# Autodesk Inventor assembly: Assembly_Matchboxscope_injectionmolded_holo
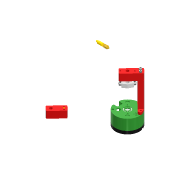
[picture p0: Inventor's stored thumbnail of the model, 180x180]
Saved by Autodesk Inventor 2022 (Build 260153000, 153)
## iProperties
Created: 2023-04-12
Part Number: Assembly_Matchboxscope_injectionmolded_holo
Document SubType Name: Assembly
Designer: diederichbenedict
Author: diederichbenedict
## Documents named in this file (11)
- C:\Users\diederichbenedict\Dropbox\Dokumente\Promotion\PROJECTS\Matchboxscope\INVENTOR\RELEASE\InjectionMolded\Assembly_Matchboxscope_injectionmolded_holo.iam
- C:\Users\diederichbenedict\Dropbox\Dokumente\Promotion\PROJECTS\Matchboxscope\INVENTOR\RELEASE\InjectionMolded\IM_Matchboxscope_base.ipt
- C:\Users\diederichbenedict\Dropbox\Dokumente\Promotion\PROJECTS\Matchboxscope\INVENTOR\RELEASE\InjectionMolded\IM_Matchboxscope_plate.ipt
- C:\Users\diederichbenedict\Dropbox\Dokumente\Promotion\PROJECTS\Matchboxscope\INVENTOR\RELEASE\InjectionMolded\Anglerfish_Cameraspacer.ipt
- C:\Users\diederichbenedict\Dropbox\Dokumente\Promotion\PROJECTS\Matchboxscope\INVENTOR\RELEASE\InjectionMolded\00_laserpointer_red.ipt
- C:\Users\diederichbenedict\Dropbox\Dokumente\Promotion\PROJECTS\Matchboxscope\INVENTOR\RELEASE\InjectionMolded\00_mk8_nozzle_0.4STEP.ipt
- C:\Users\diederichbenedict\Dropbox\Dokumente\Promotion\PROJECTS\Matchboxscope\INVENTOR\RELEASE\InjectionMolded\IM_Matchboxscope_Laserholder.ipt
- C:\Users\diederichbenedict\Dropbox\Dokumente\Promotion\PROJECTS\Matchboxscope\INVENTOR\RELEASE\InjectionMolded\IM_Matchboxscope_Laserholder_2.ipt
- C:\Users\diederichbenedict\Dropbox\Dokumente\Promotion\PROJECTS\Matchboxscope\INVENTOR\RELEASE\InjectionMolded\IM_Lensholder.ipt
- C:\Users\diederichbenedict\Documents\Inventor\Content Center Files\R2022\de-DE\DIN 912\DIN 912 - M3 x 0.5 x 16 x 14.75.ipt
- C:\Users\diederichbenedict\Dropbox\Dokumente\Promotion\PROJECTS\Matchboxscope\INVENTOR\RELEASE\InjectionMolded\IM_Matchboxscope_Laserholder_M12.ipt
## Components (14 placed, 10 different names)
1. IM_Matchboxscope_base:1 — Passend:1, Passend:2, Fluchtend:1, Fluchtend:2, Einfügen:9, Passend:3
2. Anglerfish_Cameraspacer:1
3. 00_laserpointer_red:2 — Einfügen:3, Passend:1
4. 00_mk8_nozzle_0.4STEP:1 — Einfügen:3, Passend:2
5. IM_Matchboxscope_Laserholder:1 — Fluchtend:1, Fluchtend:2, Fluchtend:3
6. IM_Matchboxscope_Laserholder_2:1 — Fluchtend:3, Einfügen:4, Einfügen:5, Einfügen:6
7. IM_Lensholder:1 — Einfügen:4, Einfügen:7, Einfügen:8
8. DIN 912 - ersetzt durch DIN EN ISO 4762 M3 x 16:1 — Einfügen:5
9. DIN 912 - ersetzt durch DIN EN ISO 4762 M3 x 16:2 — Einfügen:6
10. DIN 912 - ersetzt durch DIN EN ISO 4762 M3 x 16:3 — Einfügen:7
11. DIN 912 - ersetzt durch DIN EN ISO 4762 M3 x 16:4 — Einfügen:8
12. DIN 912 - ersetzt durch DIN EN ISO 4762 M3 x 16:5
13. IM_Matchboxscope_plate:1 — Einfügen:9, Passend:3
14. IM_Matchboxscope_Laserholder_M12:1
## Relationships (13: Insert 7, Mate 3, Flush 3)
- Einfügen:3 [Insert] (2 mm): 00_laserpointer_red:2 ↔ 00_mk8_nozzle_0.4STEP:1
- Passend:1 [Mate]: IM_Matchboxscope_base:1 ↔ 00_laserpointer_red:2
- Passend:2 [Mate] (50 mm): IM_Matchboxscope_base:1 ↔ 00_mk8_nozzle_0.4STEP:1
- Fluchtend:1 [Flush]: IM_Matchboxscope_base:1 ↔ IM_Matchboxscope_Laserholder:1
- Fluchtend:2 [Flush]: IM_Matchboxscope_base:1 ↔ IM_Matchboxscope_Laserholder:1
- Fluchtend:3 [Flush]: IM_Matchboxscope_Laserholder:1 ↔ IM_Matchboxscope_Laserholder_2:1
- Einfügen:4 [Insert] (7 mm): IM_Matchboxscope_Laserholder_2:1 ↔ IM_Lensholder:1
- Einfügen:5 [Insert]: IM_Matchboxscope_Laserholder_2:1 ↔ DIN 912 - ersetzt durch DIN EN ISO 4762 M3 x 16:1
- Einfügen:6 [Insert]: IM_Matchboxscope_Laserholder_2:1 ↔ DIN 912 - ersetzt durch DIN EN ISO 4762 M3 x 16:2
- Einfügen:7 [Insert]: IM_Lensholder:1 ↔ DIN 912 - ersetzt durch DIN EN ISO 4762 M3 x 16:3
- Einfügen:8 [Insert]: IM_Lensholder:1 ↔ DIN 912 - ersetzt durch DIN EN ISO 4762 M3 x 16:4
- Einfügen:9 [Insert]: IM_Matchboxscope_base:1 ↔ IM_Matchboxscope_plate:1
- Passend:3 [Mate]: IM_Matchboxscope_base:1 ↔ IM_Matchboxscope_plate:1
